# Autodesk Inventor assembly: SC 0610CKP4
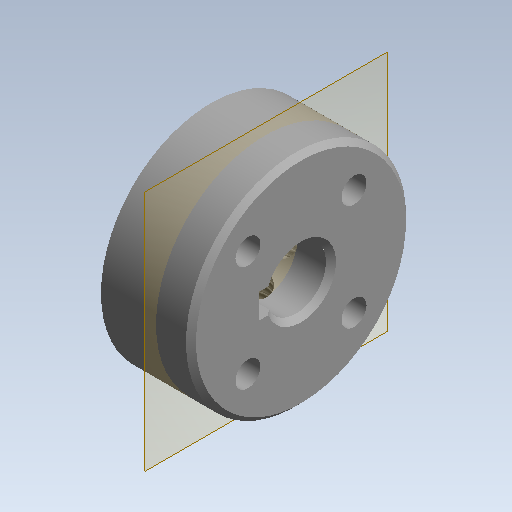
[picture p0: Inventor's stored thumbnail of the model, 512x512]
Saved by Autodesk Inventor 2021 (Build 250183000, 183)
## iProperties
Part Number: SC 0610CKP4
Catalog Web Link: www.cadenas.de
Description: SC- Black (Steel S45C)-
Vendor: IWATA
Document SubType Name: Assembly
Designer: partserver
Manufacturer: IWATA
Mass: 2.69428 g
Surface Area: 21.2219 cm^2
Volume: 2.69428 cm^3
Density: 1 g/cm^3
Category: PARTsolutions
Company: IWATA
PSOL_IDENT_0: {$CADENAS_DATA\23d-libs\iwata\standard_set_collars\with_key_groove_type\with_key_groove_type_and_4_h
PSOL_IDENT_1: oles\sc_ckp4_asmtab.prj},183 {VTYP=3D},{STYP=ASSTAB},{NB=SC 0610CKP4},{LINA=SC 0610CKP4},{NN=SC- Bla
PSOL_IDENT_2: ck (Steel S45C)},{DATE=07.01.2020 22:57:22},{GEOMDATE=15.10.2008},{VERSION=},{LINEID=20},{WBVAR=},{W
PSOL_IDENT_3: BNUMERIC=}  {NB=SC 0610CKP4},{LINA=SC 0610CKP4},{KT=DUMMY},{MAT=Steel,Black},{B=6},{L=10},{D=22},{F=
PSOL_IDENT_4: 2.5},{G=7.2},{S=4.5},{PCD=15},{M=M4 x 4},{ORDERNUMBER=SC 0610CKP4},{SMX=C},{C=0.5},{NDM=4},{KDM=3.24
PSOL_IDENT_5: 2},{H=4},{PPATH=../../standard_set_collars/../with_key_groove_type/with_key_groove_type_and_4_holes/
PSOL_IDENT_6: assemblies/ssetc_4hffwkgt_asmtpl.prj}
NB: SC 0610CKP4
NN: SC- Black (Steel S45C)
NBSYN: $ORDERNUMBER.
LINA: SC 0610CKP4
CATALOG: IWATA MFG. CO., LTD
MAT: Steel,Black
B: 6
L: 10
D: 22
F: 2.5
G: 7.2
S: 4.5
PCD: 15
M: M4 x 4
ORDERNUMBER: SC 0610CKP4
SUPPLIER: IWATA
ARTICLENO: SC 0610CKP4
BOMINFO: SC 0610CKP4
CREATOR: CADENAS GmbH
Title: SC 0610CKP4
Author: Cadenas PARTsolutions
## Documents named in this file (2)
- C:\Users\avi41\Desktop\Robot Arm\CAD_files\SC 0610CKP4.iam
- C:\Users\avi41\Desktop\Robot Arm\CAD_files\SC  0610CKP4.ipt
## Components (1 placed, 1 different names)
1. SC  0610CKP4:1 — Flush:1
## Relationships (1: Flush 1)
- Flush:1 (-3.5 mm): SC  0610CKP4:1
